# Autodesk Inventor assembly: stator-assembly
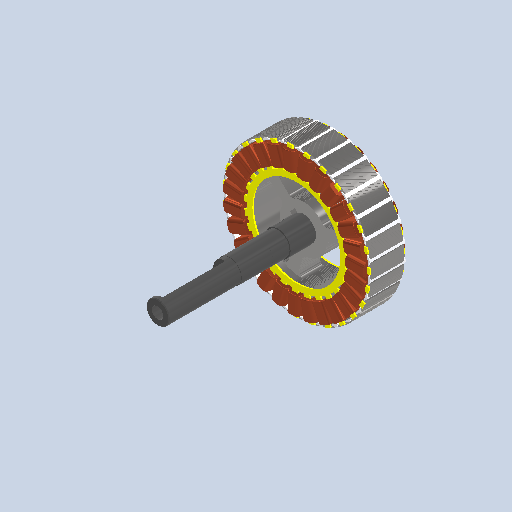
[picture p0: Inventor's stored thumbnail of the model, 512x512]
Saved by Autodesk Inventor 2022 (Build 260153000, 153)
## iProperties
Created: 2025-01-12
Part Number: stator-assembly
Document SubType Name: Assembly
Designer: Home
Author: Home
## Documents named in this file (8)
- D:\YandexDisk\Voltbro\xSets\components\HubWheel-10\stator-assembly.iam
- D:\YandexDisk\Voltbro\xSets\components\HubWheel-10\stator-sheet.ipt
- D:\YandexDisk\Voltbro\xSets\components\HubWheel-10\stator-sheet-mnt.ipt
- D:\YandexDisk\Voltbro\xSets\components\HubWheel-10\copper-wire.ipt
- D:\YandexDisk\Voltbro\xSets\components\HubWheel-10\stator-sheet-pet.ipt
- D:\YandexDisk\Voltbro\xSets\components\HubWheel-10\stator-sheet-lock.ipt
- D:\YandexDisk\Voltbro\xSets\components\HubWheel-10\shaft.ipt
- D:\YandexDisk\Voltbro\xSets\components\HubWheel-10\components\key-5x5x12.ipt
## Components (104 placed, 7 different names)
1. stator-sheet-pet:1 — Insert:3, Flush:4, Mate:6
2. stator-sheet-pet:2 — Insert:4, Flush:3
3. shaft:1 — Insert:5, Insert:6, Mate:9
4. key-5x5x12:1 — Insert:6, Mate:9, Angle:1
5. stator-sheet:1 — Insert:4, Mate:7, Mate:8, Flush:5
6. stator-sheet:2
7. stator-sheet:3 — Flush:3
8. stator-sheet:4
9. stator-sheet:5
10. stator-sheet:6
11. stator-sheet:7
12. stator-sheet:8 — Insert:2, Flush:2
13. stator-sheet-mnt:1 — Insert:2, Flush:2, Insert:5, Angle:1
14. stator-sheet-mnt:2
15. stator-sheet-mnt:3
16. stator-sheet-mnt:4
17. stator-sheet-mnt:5
18. stator-sheet-mnt:6
19. stator-sheet-mnt:7
20. stator-sheet-mnt:8
21. stator-sheet-mnt:9
22. stator-sheet-mnt:10
23. stator-sheet-mnt:11
24. stator-sheet-mnt:12
25. stator-sheet-mnt:13
26. stator-sheet-mnt:14
27. stator-sheet-mnt:15
28. stator-sheet-mnt:16
29. stator-sheet-mnt:17
30. stator-sheet-mnt:18
31. stator-sheet-mnt:19
32. stator-sheet-mnt:20
33. stator-sheet-mnt:21
34. stator-sheet-mnt:22
35. stator-sheet-mnt:23
36. stator-sheet-mnt:24
37. stator-sheet-mnt:25
38. stator-sheet-mnt:26
39. stator-sheet-mnt:27
40. stator-sheet-mnt:28
41. stator-sheet-mnt:29
42. stator-sheet-mnt:30 — Mate:5, Insert:1, Flush:1
43. stator-sheet:19 — Insert:1
44. stator-sheet:20
45. stator-sheet:21
46. stator-sheet:22
47. stator-sheet:23
48. stator-sheet:24 — Flush:4
49. stator-sheet:25 — Mate:1, Mate:3
50. stator-sheet:26 — Flush:1, Insert:3
51. copper-wire:1 — Mate:1, Mate:6
52. copper-wire:2
53. copper-wire:3
54. copper-wire:4
55. copper-wire:5
56. copper-wire:6
57. copper-wire:7
58. copper-wire:8
59. copper-wire:9
60. copper-wire:10
61. copper-wire:11
62. copper-wire:12
63. copper-wire:13
64. copper-wire:14
65. copper-wire:15
66. copper-wire:16
67. copper-wire:17
68. copper-wire:18
69. copper-wire:19
70. copper-wire:20
71. copper-wire:21
72. copper-wire:22
73. copper-wire:23
74. copper-wire:24
75. copper-wire:25
76. copper-wire:26
77. copper-wire:27
78. stator-sheet-lock:1 — Mate:7, Mate:8, Flush:5
79. stator-sheet-lock:2
80. stator-sheet-lock:3
81. stator-sheet-lock:4
82. stator-sheet-lock:5
83. stator-sheet-lock:6
84. stator-sheet-lock:7
85. stator-sheet-lock:8
86. stator-sheet-lock:9
87. stator-sheet-lock:10
88. stator-sheet-lock:11
89. stator-sheet-lock:12
90. stator-sheet-lock:13
91. stator-sheet-lock:14
92. stator-sheet-lock:15
93. stator-sheet-lock:16
94. stator-sheet-lock:17
95. stator-sheet-lock:18
96. stator-sheet-lock:19
97. stator-sheet-lock:20
98. stator-sheet-lock:21
99. stator-sheet-lock:22
100. stator-sheet-lock:23
101. stator-sheet-lock:24
102. stator-sheet-lock:25
103. stator-sheet-lock:26
104. stator-sheet-lock:27
## Component patterns: (8 elements, first: stator-sheet:1), (30 elements, first: stator-sheet-mnt:1), (8 elements, first: stator-sheet:19), (27 elements, first: copper-wire:1), (27 elements, first: stator-sheet-lock:1)
## Relationships (19: Mate 7, Insert 6, Flush 5, Angle 1)
- Mate:1: stator-sheet:25 ↔ copper-wire:1
- Mate:3: stator-sheet:25
- Mate:5: stator-sheet-mnt:30
- Insert:1: stator-sheet-mnt:30 ↔ stator-sheet:19
- Flush:1: stator-sheet-mnt:30 ↔ stator-sheet:26
- Insert:2: stator-sheet:8 ↔ stator-sheet-mnt:1
- Flush:2: stator-sheet:8 ↔ stator-sheet-mnt:1
- Insert:3: stator-sheet-pet:1 ↔ stator-sheet:26
- Insert:4: stator-sheet-pet:2 ↔ stator-sheet:1
- Flush:3: stator-sheet-pet:2 ↔ stator-sheet:3
- Flush:4: stator-sheet-pet:1 ↔ stator-sheet:24
- Mate:6: stator-sheet-pet:1 ↔ copper-wire:1
- Mate:7: stator-sheet:1 ↔ stator-sheet-lock:1
- Mate:8: stator-sheet:1 ↔ stator-sheet-lock:1
- Flush:5 (-0.5 mm): stator-sheet:1 ↔ stator-sheet-lock:1
- Insert:5: shaft:1 ↔ stator-sheet-mnt:1
- Insert:6: shaft:1 ↔ key-5x5x12:1
- Mate:9: shaft:1 ↔ key-5x5x12:1
- Angle:1 (0 deg): key-5x5x12:1 ↔ stator-sheet-mnt:1
